# Autodesk Inventor assembly: DiveTrain_FullAssembly
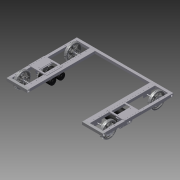
[picture p0: Inventor's stored thumbnail of the model, 180x180]
Saved by Autodesk Inventor 2012 (Build 160160000, 160)
## iProperties
Created: 2012-01-07
Part Number: DiveTrain_FullAssembly
Document SubType Name: Assembly
Designer: JesseK
Mass: 11119.1 g
Surface Area: 16891.4 cm^2
Volume: 4011.54 cm^3
Density: 2.77177 g/cm^3
Author: JesseK
## Documents named in this file (7)
- C:\Users\William\Dropbox\Robotics\CAD\team1885frc\Robot2012\DriveTrain\DiveTrain_FullAssembly.iam
- C:\Users\William\Dropbox\Robotics\CAD\team1885frc\Robot2012\DriveTrain\DriveTrain_FrameAssembly.iam
- C:\Users\William\Dropbox\Robotics\CAD\team1885frc\AndyMark\CIMpleBox\CIMple Box.iam
- C:\Users\William\Dropbox\Robotics\CAD\team1885frc\Robot2012\DriveTrain\DriveTrain_MotorMountSpacer.ipt
- C:\Users\William\Dropbox\Robotics\CAD\team1885frc\Robot2012\DriveTrain\WheelAssembly.iam
- C:\Users\William\Dropbox\Robotics\CAD\team1885frc\Robot2012\DriveTrain\DriveAxle.ipt
- C:\Users\William\Dropbox\Robotics\CAD\team1885frc\Hardware\Sprockets\Sprocket_Num25_14T_0.5bore.ipt
## Components (19 placed, 6 different names)
1. DriveTrain_FrameAssembly:1 [sub-assembly] — Mate:1, Mate:2, Mate:3, Mate:4, Mate:5, Mate:9, Flush:1, Mate:14, Flush:3, Mate:15, Flush:4, Mate:16, Flush:5, Mate:17, Mate:18, Mate:19, Mate:20
2. WheelAssembly:1 [sub-assembly] — Mate:1, Flush:2
3. CIMple Box:1 [sub-assembly] — Mate:6, Mate:7, Mate:8, Mate:10, Mate:11, Mate:12
4. DriveTrain_MotorMountSpacer:1 — Mate:2, Mate:5, Mate:6
5. DriveTrain_MotorMountSpacer:2 — Mate:3, Mate:4, Mate:7, Mate:8
6. DriveAxle:1 — Mate:9, Flush:1
7. DriveAxle:2 — Mate:15, Flush:4, Mate:30
8. DriveAxle:3 — Mate:14, Flush:3, Mate:28
9. DriveAxle:4 — Mate:16, Flush:5, Mate:29
10. Sprocket_Num25_14T_0.5bore:1 — Mate:10, Mate:11, Flush:2, Mate:13
11. Sprocket_Num25_14T_0.5bore:2 — Mate:12, Mate:13, Flush:6
12. Sprocket_Num25_14T_0.5bore:3 — Mate:25, Mate:27, Flush:8
13. Sprocket_Num25_14T_0.5bore:4 — Mate:24, Mate:26, Mate:27, Flush:7
14. CIMple Box:2 [sub-assembly] — Mate:21, Mate:22, Mate:23, Mate:24, Mate:25, Mate:26
15. WheelAssembly:2 [sub-assembly] — Mate:28, Flush:6
16. WheelAssembly:3 [sub-assembly] — Mate:29, Flush:8
17. WheelAssembly:4 [sub-assembly] — Mate:30, Flush:7
18. DriveTrain_MotorMountSpacer:3 — Mate:17, Mate:19, Mate:21, Mate:22
19. DriveTrain_MotorMountSpacer:4 — Mate:18, Mate:20, Mate:23
## Relationships (38: Mate 30, Flush 8)
- Mate:1: DriveTrain_FrameAssembly:1 ↔ WheelAssembly:1
- Mate:2: DriveTrain_FrameAssembly:1 ↔ DriveTrain_MotorMountSpacer:1
- Mate:3: DriveTrain_FrameAssembly:1 ↔ DriveTrain_MotorMountSpacer:2
- Mate:4: DriveTrain_FrameAssembly:1 ↔ DriveTrain_MotorMountSpacer:2
- Mate:5: DriveTrain_FrameAssembly:1 ↔ DriveTrain_MotorMountSpacer:1
- Mate:6: CIMple Box:1 ↔ DriveTrain_MotorMountSpacer:1
- Mate:7: CIMple Box:1 ↔ DriveTrain_MotorMountSpacer:2
- Mate:8: CIMple Box:1 ↔ DriveTrain_MotorMountSpacer:2
- Mate:9: DriveTrain_FrameAssembly:1 ↔ DriveAxle:1
- Flush:1 (-9.525 mm): DriveTrain_FrameAssembly:1 ↔ DriveAxle:1
- Mate:10: CIMple Box:1 ↔ Sprocket_Num25_14T_0.5bore:1
- Mate:11: CIMple Box:1 ↔ Sprocket_Num25_14T_0.5bore:1
- Flush:2: WheelAssembly:1 ↔ Sprocket_Num25_14T_0.5bore:1
- Mate:12: CIMple Box:1 ↔ Sprocket_Num25_14T_0.5bore:2
- Mate:13: Sprocket_Num25_14T_0.5bore:1 ↔ Sprocket_Num25_14T_0.5bore:2
- Mate:14: DriveTrain_FrameAssembly:1 ↔ DriveAxle:3
- Flush:3 (-9.525 mm): DriveTrain_FrameAssembly:1 ↔ DriveAxle:3
- Mate:15: DriveTrain_FrameAssembly:1 ↔ DriveAxle:2
- Flush:4 (-9.525 mm): DriveTrain_FrameAssembly:1 ↔ DriveAxle:2
- Mate:16: DriveTrain_FrameAssembly:1 ↔ DriveAxle:4
- Flush:5 (-9.525 mm): DriveTrain_FrameAssembly:1 ↔ DriveAxle:4
- Mate:17: DriveTrain_FrameAssembly:1 ↔ DriveTrain_MotorMountSpacer:3
- Mate:18: DriveTrain_FrameAssembly:1 ↔ DriveTrain_MotorMountSpacer:4
- Mate:19: DriveTrain_FrameAssembly:1 ↔ DriveTrain_MotorMountSpacer:3
- Mate:20: DriveTrain_FrameAssembly:1 ↔ DriveTrain_MotorMountSpacer:4
- Mate:21: CIMple Box:2 ↔ DriveTrain_MotorMountSpacer:3
- Mate:22: CIMple Box:2 ↔ DriveTrain_MotorMountSpacer:3
- Mate:23: CIMple Box:2 ↔ DriveTrain_MotorMountSpacer:4
- Mate:24: Sprocket_Num25_14T_0.5bore:4 ↔ CIMple Box:2
- Mate:25: Sprocket_Num25_14T_0.5bore:3 ↔ CIMple Box:2
- Mate:26: Sprocket_Num25_14T_0.5bore:4 ↔ CIMple Box:2
- Mate:27: Sprocket_Num25_14T_0.5bore:3 ↔ Sprocket_Num25_14T_0.5bore:4
- Mate:28: DriveAxle:3 ↔ WheelAssembly:2
- Flush:6: Sprocket_Num25_14T_0.5bore:2 ↔ WheelAssembly:2
- Mate:29: DriveAxle:4 ↔ WheelAssembly:3
- Mate:30: DriveAxle:2 ↔ WheelAssembly:4
- Flush:7: Sprocket_Num25_14T_0.5bore:4 ↔ WheelAssembly:4
- Flush:8: Sprocket_Num25_14T_0.5bore:3 ↔ WheelAssembly:3
